# Autodesk Inventor assembly: the robot
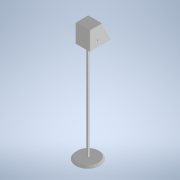
[picture p0: Inventor's stored thumbnail of the model, 180x180]
Saved by Autodesk Inventor 2022 (Build 260153000, 153)
## iProperties
Created: 2021-07-21
Part Number: the robot
Document SubType Name: Assembly
Designer: fanam
Author: fanam
## Documents named in this file (4)
- C:\Users\fanam\OneDrive\سطح المكتب\the robot.iam
- C:\Users\fanam\OneDrive\سطح المكتب\Part3 top.ipt
- C:\Users\fanam\OneDrive\سطح المكتب\the head (top).ipt
- C:\Users\fanam\OneDrive\سطح المكتب\the mid.ipt
## Components (3 placed, 3 different names)
1. Part3 top:1 — Rigid:1
2. the head (top):1 — Rotational:1
3. the mid:1 — Rigid:1, Rotational:1
## Relationships (2: WeldJoint 1, RevoluteJoint 1)
- Rigid:1 [WeldJoint]: Part3 top:1 ↔ the mid:1
- Rotational:1 [RevoluteJoint]: the head (top):1 ↔ the mid:1
